# Autodesk Inventor assembly: EnsambleMecanismoEnsayo2
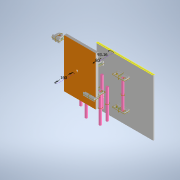
[picture p0: Inventor's stored thumbnail of the model, 180x180]
Saved by Autodesk Inventor 2021 (Build 250183000, 183)
## iProperties
Created: 2021-04-17
Part Number: EnsambleMecanismoEnsayo2
Document SubType Name: Assembly
Designer: GABRIEL LOL
Author: GABRIEL LOL
## Documents named in this file (8)
- J:\PAI\Proyecto_PAI_2021\01 CAD\EnsambleMecanismoEnsayo2.iam
- J:\PAI\Proyecto_PAI_2021\01 CAD\PasadorPivotePreliminar.ipt
- J:\PAI\Proyecto_PAI_2021\01 CAD\PasadorPreliminar.ipt
- J:\PAI\Proyecto_PAI_2021\01 CAD\ApoyoRotatorioPreliminar.ipt
- J:\PAI\Proyecto_PAI_2021\01 CAD\PistaEslabonPreliminar.ipt
- J:\PAI\Proyecto_PAI_2021\01 CAD\SoporteBaseElevacion.ipt
- J:\PAI\Proyecto_PAI_2021\01 CAD\BaseExtrusion.ipt
- J:\PAI\Proyecto_PAI_2021\01 CAD\PisoDeEnsayoIgnorar.ipt
## Components (21 placed, 7 different names)
1. ApoyoRotatorioPreliminar:3 — Mate:2, Mate:7, Flush:3, Mate:16
2. ApoyoRotatorioPreliminar:4 — Mate:1, Mate:5, Mate:7, Flush:2, Flush:3, Flush:4, Mate:21, Mate:22
3. PasadorPivotePreliminar:3 — Mate:16
4. PasadorPivotePreliminar:4 — Mate:5
5. PasadorPreliminar:2
6. PistaEslabonPreliminar:1 — Mate:20, Mate:23, Mate:24, Transitional:3, Transitional:4, Flush:37
7. PistaEslabonPreliminar:2 — Mate:19, Mate:21, Mate:22, Mate:23, Mate:24, Flush:36
8. SoporteBaseElevacion:1 — Mate:8, Mate:9, Mate:10, Mate:51, Mate:52, Flush:33, Flush:34, Mate:53
9. BaseExtrusion:1 — Mate:8, Mate:9, Mate:10
10. PisoDeEnsayoIgnorar:1 — Mate:1, Mate:2, Flush:2, Flush:4, Mate:19, Mate:20
11. PasadorPreliminar:6 — Transitional:3, Transitional:4
12. PasadorPreliminar:8
13. PasadorPreliminar:11
14. PasadorPreliminar:14
15. PasadorPreliminar:15 — Transitional:5, Transitional:6, Flush:31
16. PasadorPivotePreliminar:5 — Mate:47
17. PasadorPivotePreliminar:6 — Mate:45, Mate:54, Flush:38
18. ApoyoRotatorioPreliminar:5 — Mate:45, Mate:53, Mate:54, Flush:38
19. ApoyoRotatorioPreliminar:6 — Mate:47, Mate:52, Flush:33, Flush:34
20. PistaEslabonPreliminar:3 — Transitional:5, Transitional:6, Flush:31, Mate:51, Flush:35, Flush:37
21. PistaEslabonPreliminar:4 — Flush:35, Flush:36
## Relationships (34: Mate 20, Flush 10, Transitional 4)
- Mate:1: ApoyoRotatorioPreliminar:4 ↔ PisoDeEnsayoIgnorar:1
- Mate:2: ApoyoRotatorioPreliminar:3 ↔ PisoDeEnsayoIgnorar:1
- Mate:5: ApoyoRotatorioPreliminar:4 ↔ PasadorPivotePreliminar:4
- Mate:7: ApoyoRotatorioPreliminar:3 ↔ ApoyoRotatorioPreliminar:4
- Mate:8: SoporteBaseElevacion:1 ↔ BaseExtrusion:1
- Mate:9: SoporteBaseElevacion:1 ↔ BaseExtrusion:1
- Mate:10: SoporteBaseElevacion:1 ↔ BaseExtrusion:1
- Flush:2: ApoyoRotatorioPreliminar:4 ↔ PisoDeEnsayoIgnorar:1
- Flush:3 (250 mm): ApoyoRotatorioPreliminar:3 ↔ ApoyoRotatorioPreliminar:4
- Flush:4 (108 mm): ApoyoRotatorioPreliminar:4 ↔ PisoDeEnsayoIgnorar:1
- Mate:16: ApoyoRotatorioPreliminar:3 ↔ PasadorPivotePreliminar:3
- Mate:19: PistaEslabonPreliminar:2 ↔ PisoDeEnsayoIgnorar:1
- Mate:20: PistaEslabonPreliminar:1 ↔ PisoDeEnsayoIgnorar:1
- Mate:21: ApoyoRotatorioPreliminar:4 ↔ PistaEslabonPreliminar:2
- Mate:22 (173.4 mm): ApoyoRotatorioPreliminar:4 ↔ PistaEslabonPreliminar:2
- Mate:23: PistaEslabonPreliminar:1 ↔ PistaEslabonPreliminar:2
- Mate:24 (-250 mm): PistaEslabonPreliminar:1 ↔ PistaEslabonPreliminar:2
- Transitional:3: PistaEslabonPreliminar:1 ↔ PasadorPreliminar:6
- Transitional:4: PistaEslabonPreliminar:1 ↔ PasadorPreliminar:6
- Mate:45: PasadorPivotePreliminar:6 ↔ ApoyoRotatorioPreliminar:5
- Mate:47: PasadorPivotePreliminar:5 ↔ ApoyoRotatorioPreliminar:6
- Transitional:5: PasadorPreliminar:15 ↔ PistaEslabonPreliminar:3
- Transitional:6: PasadorPreliminar:15 ↔ PistaEslabonPreliminar:3
- Flush:31: PasadorPreliminar:15 ↔ PistaEslabonPreliminar:3
- Mate:51: SoporteBaseElevacion:1 ↔ PistaEslabonPreliminar:3
- Mate:52: SoporteBaseElevacion:1 ↔ ApoyoRotatorioPreliminar:6
- Flush:33: SoporteBaseElevacion:1 ↔ ApoyoRotatorioPreliminar:6
- Flush:34 (105 mm): SoporteBaseElevacion:1 ↔ ApoyoRotatorioPreliminar:6
- Mate:53: SoporteBaseElevacion:1 ↔ ApoyoRotatorioPreliminar:5
- Flush:35: PistaEslabonPreliminar:3 ↔ PistaEslabonPreliminar:4
- Flush:36: PistaEslabonPreliminar:2 ↔ PistaEslabonPreliminar:4
- Flush:37: PistaEslabonPreliminar:1 ↔ PistaEslabonPreliminar:3
- Mate:54: PasadorPivotePreliminar:6 ↔ ApoyoRotatorioPreliminar:5
- Flush:38: PasadorPivotePreliminar:6 ↔ ApoyoRotatorioPreliminar:5
